# Autodesk Inventor assembly: Battery box
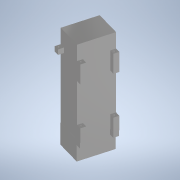
[picture p0: Inventor's stored thumbnail of the model, 180x180]
Saved by Autodesk Inventor 2022.2 (Build 262287000, 287)
## iProperties
Created: 2022-04-11
Part Number: Battery box
Document SubType Name: Assembly
Designer: foriw
Author: foriw
## Documents named in this file (3)
- H:\inventor ting\Mekatronik beercart git\Beercart CAD\Workspaces\Workspace\Battery box.iam
- H:\inventor ting\Mekatronik beercart git\Beercart CAD\Workspaces\Workspace\Batteriholder v1\Component1.ipt
- H:\inventor ting\Mekatronik beercart git\Beercart CAD\Workspaces\Workspace\Batteriholder v1\Part4.ipt
## Components (3 placed, 2 different names)
1. Component1:1
2. Part4:1
3. Component1:2
## Relationships (5: Mate 4, Angle 1)
- [Angle] (0 deg): Part4:1 ↔ Component1:2
- [Mate]: Part4:1 ↔ Component1:2
- [Mate]: Part4:1 ↔ Component1:2
- [Mate]: Part4:1 ↔ Component1:2
- [Mate]: Component1:1 ↔ Part4:1
